# Autodesk Inventor assembly: flute
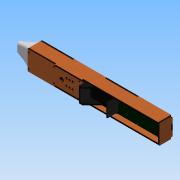
[picture p0: Inventor's stored thumbnail of the model, 180x180]
Saved by Autodesk Inventor 2015 (Build 190159000, 159)
## iProperties
Created: 2015-12-28
Part Number: flute
Document SubType Name: Assembly
Designer: Gregwar
Author: Gregwar
## Documents named in this file (8)
- C:\Users\Gregwar\Desktop\eFlute\3d\v1\flute.iam
- C:\Users\Gregwar\Desktop\eFlute\3d\v1\electronics.ipt
- C:\Users\Gregwar\Desktop\eFlute\3d\v1\bec.ipt
- C:\Users\Gregwar\Desktop\eFlute\3d\v1\top.ipt
- C:\Users\Gregwar\Desktop\eFlute\3d\v1\side.ipt
- C:\Users\Gregwar\Desktop\eFlute\3d\v1\bottom.ipt
- C:\Users\Gregwar\Desktop\eFlute\3d\v1\bottom_renfort.ipt
- C:\Users\Gregwar\Desktop\eFlute\3d\v1\connectors.ipt
## Components (8 placed, 7 different names)
1. electronics:1 — Placage:1, Placage:2, Placage:3
2. bec:1 — Placage:1, Placage:2, Placage:3, Placage:4, Placage:5, Placage:6, Placage:10, Placage:11
3. top:1 — Placage:4, Placage:5, Placage:6, Placage:7, Affleurement:1, Affleurement:2, Placage:8, Affleurement:3, Affleurement:4, Placage:14, Affleurement:6, Placage:15
4. side:1 — Placage:7, Affleurement:1, Affleurement:2
5. side:2 — Placage:8, Affleurement:3, Affleurement:4, Placage:9
6. bottom:1 — Placage:9, Placage:10, Placage:11, Placage:12, Affleurement:5, Placage:13
7. bottom_renfort:1 — Placage:12, Affleurement:5, Placage:13
8. connectors:1 — Placage:14, Affleurement:6, Placage:15
## Relationships (21: Mate 15, Flush 6)
- Placage:1 [Mate]: electronics:1 ↔ bec:1
- Placage:2 [Mate]: electronics:1 ↔ bec:1
- Placage:3 [Mate]: electronics:1 ↔ bec:1
- Placage:4 [Mate]: bec:1 ↔ top:1
- Placage:5 [Mate]: bec:1 ↔ top:1
- Placage:6 [Mate]: bec:1 ↔ top:1
- Placage:7 [Mate]: top:1 ↔ side:1
- Affleurement:1 [Flush]: top:1 ↔ side:1
- Affleurement:2 [Flush]: top:1 ↔ side:1
- Placage:8 [Mate]: top:1 ↔ side:2
- Affleurement:3 [Flush]: top:1 ↔ side:2
- Affleurement:4 [Flush]: top:1 ↔ side:2
- Placage:9 [Mate]: side:2 ↔ bottom:1
- Placage:10 [Mate]: bec:1 ↔ bottom:1
- Placage:11 [Mate]: bec:1 ↔ bottom:1
- Placage:12 [Mate]: bottom:1 ↔ bottom_renfort:1
- Affleurement:5 [Flush]: bottom:1 ↔ bottom_renfort:1
- Placage:13 [Mate]: bottom:1 ↔ bottom_renfort:1
- Placage:14 [Mate]: top:1 ↔ connectors:1
- Affleurement:6 [Flush]: top:1 ↔ connectors:1
- Placage:15 [Mate]: top:1 ↔ connectors:1
